# Autodesk Inventor assembly: Assembly2
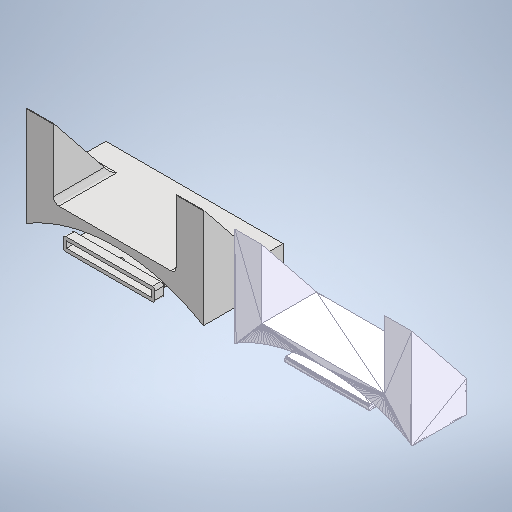
[picture p0: Inventor's stored thumbnail of the model, 512x512]
Saved by Autodesk Inventor 2025.1 (Build 291241000, 241)
## iProperties
Created: 2026-03-14
Part Number: Assembly2
Document SubType Name: Assembly
Designer: User
Author: User
## Documents named in this file (4)
- D:\One Drive\OneDrive - Politeknik Sultan Salahuddin Abdul Aziz Shah\Documents\Inventor\RobosotPSA\Assembly2.iam
- D:\One Drive\OneDrive - Politeknik Sultan Salahuddin Abdul Aziz Shah\Documents\Inventor\FAC_RC_Car\DC Geared Motor RB350100-0A101R\sumo soccer.ipt
- D:\One Drive\OneDrive - Politeknik Sultan Salahuddin Abdul Aziz Shah\Documents\Inventor\RobosotPSA\DuplicateSumoSoccer.ipt
- D:\One Drive\OneDrive - Politeknik Sultan Salahuddin Abdul Aziz Shah\Documents\Inventor\RobosotPSA\spacer.ipt
## Components (3 placed, 3 different names)
1. DuplicateSumoSoccer:1 — Flush:1, Flush:2, Flush:3, Flush:4
2. sumo soccer:1 — Flush:2, Flush:3
3. spacer:1 — Flush:4
## Relationships (4: Flush 4)
- Flush:1: DuplicateSumoSoccer:1
- Flush:2: DuplicateSumoSoccer:1 ↔ sumo soccer:1
- Flush:3: DuplicateSumoSoccer:1 ↔ sumo soccer:1
- Flush:4: DuplicateSumoSoccer:1 ↔ spacer:1
